# Autodesk Inventor assembly: Slew Bearing v2 v18
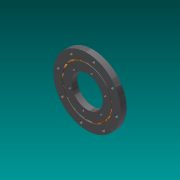
[picture p0: Inventor's stored thumbnail of the model, 180x180]
Saved by Autodesk Inventor 2020.3 (Build 243373000, 373)
## iProperties
Created: 2020-05-24
Part Number: Slew Bearing v2 v18
Document SubType Name: Assembly
Designer: Administrator
Title: Slew Bearing v2 v18 v9
Author: Administrator
## Documents named in this file (5)
- C:\Users\Svend\OneDrive\Documents\GitHub\BeerMinder\3D-model\bearings\slew bearing 80 mm\Slew Bearing 80mm.iam
- C:\Users\Svend\OneDrive\Documents\GitHub\BeerMinder\3D-model\bearings\slew bearing 80 mm\Rolls A 80mm.ipt
- C:\Users\Svend\OneDrive\Documents\GitHub\BeerMinder\3D-model\bearings\slew bearing 80 mm\Race Outer 80mm.ipt
- C:\Users\Svend\OneDrive\Documents\GitHub\BeerMinder\3D-model\bearings\slew bearing 80 mm\Rolls B 80mm.ipt
- C:\Users\Svend\OneDrive\Documents\GitHub\BeerMinder\3D-model\bearings\slew bearing 80 mm\Race Inner 80mm.iam
## Components (4 placed, 4 different names)
1. Rolls A 80mm:1 — Mate:2, Mate:3
2. Rolls B:1 — Mate:4, Mate:5, Angle:1
3. Race Outer 80mm:1 — Mate:1, Mate:2, Mate:3, Mate:4, Mate:5, Angle:1, Mate:6
4. Race Inner 80mm:1 [sub-assembly] — Mate:1, Mate:6
## Relationships (7: Mate 6, Angle 1)
- Mate:1: Race Outer 80mm:1 ↔ Race Inner 80mm:1
- Mate:2: Rolls A 80mm:1 ↔ Race Outer 80mm:1
- Mate:3: Rolls A 80mm:1 ↔ Race Outer 80mm:1
- Mate:4: Rolls B:1 ↔ Race Outer 80mm:1
- Mate:5: Rolls B:1 ↔ Race Outer 80mm:1
- Angle:1 (59.5 deg): Rolls B:1 ↔ Race Outer 80mm:1
- Mate:6: Race Outer 80mm:1 ↔ Race Inner 80mm:1
